# Autodesk Inventor assembly: ext_roof bar assembly
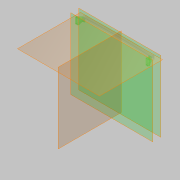
[picture p0: Inventor's stored thumbnail of the model, 180x180]
Saved by Autodesk Inventor 2021 (Build 250183000, 183)
## iProperties
Created: 2017-07-25
Part Number: ext_roof bar assembly
Description: SolidWorks IGES file using analytic representation for surfaces
Document SubType Name: Assembly
Designer: Watchdog
Sending System: SolidWorks 2016
Preprocessor: SolidWorks 2016
Minimum Resolution: 0.0
Sending System Product ID: Assem2
Receiving System Product ID: Assem2
Sent Units: Millimeter
Translation Standard: IGES 5.3
Model Creation Time: 2017-07-25
Title: C:\Users\Sandy\Documents\Solidworks parts\lupo\roof bar assembly.IGS
Author: Sandy
## Documents named in this file (5)
- C:\Users\Watchdog\OneDrive - Flinders\Advn Mech Design Shared\6_Development\2_Design\inventor\support\roof_bar\ext_roof bar assembly.iam
- C:\Users\Watchdog\OneDrive - Flinders\Advn Mech Design Shared\6_Development\2_Design\inventor\support\roof_bar\ext_roof bars.ipt
- C:\Users\Watchdog\OneDrive - Flinders\Advn Mech Design Shared\6_Development\2_Design\inventor\support\roof_bar\ext_roof bar stand.ipt
- C:\Users\Watchdog\OneDrive - Flinders\Advn Mech Design Shared\6_Development\2_Design\inventor\support\roof_bar\ext_socket head cap screw_ai_HX-SHCS 0.19-32x1.375x1-N.ipt
- C:\Users\Watchdog\OneDrive - Flinders\Advn Mech Design Shared\6_Development\2_Design\inventor\support\roof_bar\ext_acorn high crown nut_61_ai_AHCNUT 0.1900-32-N.ipt
## Components (7 placed, 4 different names)
1. ext_roof bars
2. ext_roof bar stand
3. ext_roof bar stand:1
4. ext_socket head cap screw_ai_HX-SHCS 0.19-32x1.375x1-N
5. ext_acorn high crown nut_61_ai_AHCNUT 0.1900-32-N
6. ext_acorn high crown nut_61_ai_AHCNUT 0.1900-32-N:1
7. ext_acorn high crown nut_61_ai_AHCNUT 0.1900-32-N:2
## Relationships (4: Flush 4)
- Flush:1 (584 mm)
- Flush:2 (127.5 mm)
- Flush:3 (350 mm)
- Flush:4 (790.5 mm)
